# Autodesk Inventor assembly: Passion-v2
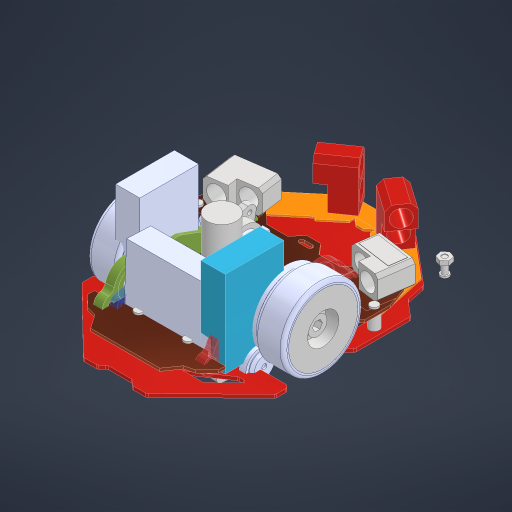
[picture p0: Inventor's stored thumbnail of the model, 512x512]
Saved by Autodesk Inventor 2023.5 (Build 275446000, 446)
## iProperties
Created: 2024-12-07
Part Number: Passion-v2
Document SubType Name: Assembly
Designer: IshiiLabHonda
Author: IshiiLabHonda
## Documents named in this file (31)
- C:\Users\IshiiLabHonda\Documents\Micromouse\Passion-v2\Inventor\Passion-v2-1\Passion-v2.iam
- C:\Users\IshiiLabHonda\Documents\Micromouse\Passion-v2\Inventor\Passion-v2-1\Readymade\Encoder-Gear_M0.3_29T.ipt
- C:\Users\IshiiLabHonda\Documents\Micromouse\Passion-v2\Inventor\Passion-v2-1\Readymade\Encoder-Gear-Spacer.ipt
- C:\Users\IshiiLabHonda\Documents\Micromouse\Passion-v2\Inventor\Passion-v2-1\Readymade\Motor-8523.ipt
- C:\Users\IshiiLabHonda\Documents\Micromouse\Passion-v2\Inventor\Passion-v2-1\Readymade\Pinion-Gear_M0.3_15T.ipt
- C:\Users\IshiiLabHonda\Documents\Micromouse\Passion-v2\Inventor\Passion-v2-1\Readymade\Spur-Gear_M0.3_71T_t2.0_D8.ipt
- C:\Users\IshiiLabHonda\Documents\Micromouse\Passion-v2\Inventor\Passion-v2-1\Readymade\Tire-MZW39-40.ipt
- C:\Users\IshiiLabHonda\Documents\Micromouse\Passion-v2\Inventor\Passion-v2-1\Readymade\Wheel_MZH131W-N2.ipt
- C:\Users\IshiiLabHonda\Documents\Micromouse\Passion-v2\Inventor\Passion-v2-1\Common\spacer_inwheel_1.1.ipt
- C:\Users\IshiiLabHonda\Documents\Micromouse\Passion-v2\Inventor\Passion-v2-1\Common\bearing_SMR63ZZ.ipt
- C:\Users\IshiiLabHonda\Documents\Micromouse\Passion-v2\Inventor\Passion-v2-1\Common\M3_bolt.ipt
- C:\Users\IshiiLabHonda\Documents\Micromouse\Passion-v2\Inventor\Passion-v2-1\Readymade\Encoder-7S-400-2MC-50-00E.ipt
- C:\Users\IshiiLabHonda\Documents\Micromouse\Passion-v2\Inventor\Passion-v2-1\Readymade\Motor-8520.ipt
- C:\Users\IshiiLabHonda\Documents\Micromouse\Passion-v2\Inventor\Passion-v2-1\Origin\encoderauxiliary.ipt
- C:\Users\IshiiLabHonda\Documents\Micromouse\Passion-v2\Inventor\Passion-v2-1\Origin\motorauxiliary.ipt
- C:\Users\IshiiLabHonda\Documents\Micromouse\Passion-v2\Inventor\Passion-v2-1\Origin\fan.ipt
- C:\Users\IshiiLabHonda\Documents\Micromouse\Passion-v2\Inventor\Passion-v2-1\Origin\motormount.ipt
- C:\Users\IshiiLabHonda\Documents\Micromouse\Passion-v2\Inventor\Passion-v2-2\Common\Li-Po_JJRC-150mAh.ipt
- C:\Users\IshiiLabHonda\Documents\Micromouse\Passion-v2\Inventor\Passion-v2-1\Origin\chassis.ipt
- C:\Users\IshiiLabHonda\Documents\Micromouse\Passion-v2\Inventor\Passion-v2-1\Origin\sensorholder_2.ipt
- C:\Users\IshiiLabHonda\Documents\Micromouse\Passion-v2\Inventor\Passion-v2-1\Origin\circuit.ipt
- C:\Users\IshiiLabHonda\Documents\Micromouse\Passion-v2\Inventor\Passion-v2-1\Common\spacer_m1.6_circuit.ipt
- C:\Users\IshiiLabHonda\Documents\Micromouse\Passion-v2\Inventor\Passion-v2-1\Common\m1.6_2_なべ小ねじ0番.ipt
- C:\Users\IshiiLabHonda\Documents\Micromouse\Passion-v2\Inventor\Passion-v2-1\Origin\sensorcircuit.ipt
- C:\Users\IshiiLabHonda\Documents\Micromouse\Passion-v2\Inventor\Passion-v2-1\Origin\sensorholder_3.ipt
- C:\Users\IshiiLabHonda\Documents\Micromouse\Passion-v2\Inventor\Passion-v2-1\Origin\fanauxiliary.ipt
- C:\Users\IshiiLabHonda\Documents\Micromouse\Passion-v2\Inventor\Passion-v2-1\Common\m1.6_3_なべ小ねじ0番.ipt
- C:\Users\IshiiLabHonda\Documents\Micromouse\Passion-v2\Inventor\Passion-v2-1\Common\m1.6_4_なべ小ねじ0番.ipt
- C:\Users\IshiiLabHonda\Documents\Micromouse\Passion-v2\Inventor\Passion-v2-1\Common\m1.6_nut.ipt
- C:\Users\IshiiLabHonda\Documents\Micromouse\Passion-v2\Inventor\Passion-v2-1\Common\m1.6_5_なべ小ねじ0番.ipt
- C:\Users\IshiiLabHonda\Documents\Micromouse\Passion-v2\Inventor\Passion-v2-1\Common\spacer-outwheel-m3-1.ipt
## Components (70 placed, 30 different names)
1. Motor-8520:1 — メイト:234, メイト:235, メイト:239
2. fan:1 — メイト:235, メイト:236, メイト:237
3. Encoder-Gear_M0.3_29T:2
4. Encoder-Gear-Spacer:2 — メイト:147
5. Motor-8523:2 — メイト:148, メイト:150, メイト:267
6. Pinion-Gear_M0.3_15T:2 — メイト:150, フラッシュ:23
7. Spur-Gear_M0.3_71T_t2.0_D8:2 — フラッシュ:23, メイト:290
8. Tire-MZW39-40:2
9. Wheel_MZH131W-N2:2
10. spacer_inwheel_1.1:2
11. bearing_SMR63ZZ:3
12. bearing_SMR63ZZ:4 — メイト:139
13. M3_bolt:2 — メイト:136, メイト:139, メイト:284
14. Encoder-7S-400-2MC-50-00E:2 — メイト:147, メイト:243, メイト:264
15. encoderauxiliary:2 — メイト:143, メイト:145, メイト:243
16. motorauxiliary:2 — メイト:140, メイト:142, メイト:148
17. motormount:2 — メイト:152, メイト:154, メイト:156, メイト:159, メイト:219, メイト:224, メイト:225, メイト:266, メイト:287, メイト:288
18. Li-Po_JJRC-150mAh:2
19. Encoder-Gear_M0.3_29T:3 — フラッシュ:25
20. Encoder-Gear-Spacer:3 — メイト:265
21. Motor-8523:3 — メイト:155, メイト:156
22. Pinion-Gear_M0.3_15T:3 — フラッシュ:24
23. Spur-Gear_M0.3_71T_t2.0_D8:3 — メイト:161, メイト:162, フラッシュ:24, フラッシュ:25, メイト:289
24. Tire-MZW39-40:3
25. Wheel_MZH131W-N2:3 — メイト:161, メイト:162
26. spacer_inwheel_1.1:3
27. bearing_SMR63ZZ:5
28. bearing_SMR63ZZ:6 — メイト:171, メイト:172
29. M3_bolt:3 — メイト:171, メイト:172, メイト:286, メイト:288
30. Encoder-7S-400-2MC-50-00E:3 — メイト:160, メイト:265, メイト:266
31. encoderauxiliary:3 — メイト:159, メイト:160, メイト:219
32. motorauxiliary:3 — メイト:152, メイト:154, メイト:155
33. motormount:3 — メイト:136, メイト:140, メイト:142, メイト:143, メイト:145, メイト:222, メイト:223, メイト:264, メイト:267, メイト:285
34. chassis:1 — メイト:177, メイト:181, メイト:182, メイト:192, メイト:195, メイト:201, メイト:206, フラッシュ:26, メイト:211, メイト:222, メイト:223, メイト:224, メイト:225, メイト:226, メイト:227, メイト:229, メイト:236, メイト:237, メイト:247, メイト:248, フラッシュ:27, メイト:255, メイト:261, メイト:263, メイト:275, メイト:278, メイト:280, メイト:281, メイト:283
35. sensorholder_2:2 — フラッシュ:27
36. sensorholder_2:4 — フラッシュ:26
37. circuit:1 — メイト:178, メイト:180, メイト:191, メイト:193, メイト:199, メイト:200, メイト:205, メイト:207, メイト:209, メイト:210, メイト:212, メイト:218, メイト:231, メイト:238, メイト:239, メイト:240, メイト:252, メイト:254, メイト:257, メイト:260, メイト:262, フラッシュ:269, フラッシュ:270, フラッシュ:273, メイト:291, フラッシュ:274
38. spacer_m1.6_circuit:1 — メイト:177, メイト:178, メイト:210
39. m1.6_2_なべ小ねじ0番:1 — メイト:180, メイト:218
40. m1.6_2_なべ小ねじ0番:2 — メイト:181, メイト:182
41. spacer_m1.6_circuit:2 — メイト:192, メイト:193, メイト:194, メイト:255
42. m1.6_2_なべ小ねじ0番:3 — メイト:191, メイト:212
43. m1.6_2_なべ小ねじ0番:4 — メイト:194, メイト:195
44. spacer_m1.6_circuit:3 — メイト:197, メイト:198, メイト:200, メイト:209, メイト:211
45. m1.6_2_なべ小ねじ0番:5 — メイト:197, メイト:199
46. m1.6_2_なべ小ねじ0番:6 — メイト:198, メイト:201
47. spacer_m1.6_circuit:4 — メイト:205
48. m1.6_2_なべ小ねじ0番:7 — メイト:207
49. m1.6_2_なべ小ねじ0番:8 — メイト:206
50. sensorcircuit:1 — メイト:247, メイト:248, メイト:271, メイト:273, メイト:274, メイト:279
51. sensorholder_3:1 — メイト:240, フラッシュ:269, フラッシュ:270
52. spacer_m1.6_circuit:5 — メイト:226, メイト:229, メイト:230
53. m1.6_2_なべ小ねじ0番:9 — メイト:230, メイト:231
54. m1.6_2_なべ小ねじ0番:10 — メイト:227, メイト:283
55. fanauxiliary:1 — メイト:234, メイト:238, メイト:252, メイト:253, メイト:256
56. m1.6_3_なべ小ねじ0番:1 — メイト:253, メイト:254
57. m1.6_3_なべ小ねじ0番:2 — メイト:256, メイト:257
58. spacer_m1.6_circuit:6 — メイト:260, メイト:261
59. m1.6_2_なべ小ねじ0番:11 — メイト:262
60. m1.6_2_なべ小ねじ0番:12 — メイト:263
61. m1.6_nut:1 — メイト:271, メイト:282
62. m1.6_4_なべ小ねじ0番:2 — メイト:273, メイト:275
63. m1.6_nut:2 — メイト:274
64. m1.6_nut:3 — メイト:278, メイト:279
65. m1.6_5_なべ小ねじ0番:1 — メイト:280, メイト:281, メイト:282
66. spacer-outwheel-m3-1:1 — メイト:284, メイト:285, メイト:290
67. spacer-outwheel-m3-1:2 — メイト:286, メイト:287, メイト:289
68. sensorholder_3:2 — フラッシュ:273, メイト:291, フラッシュ:274
69. Li-Po_JJRC-150mAh:3
70. Li-Po_JJRC-150mAh:4
## Relationships (133: Mate 118, Flush 14, Tangent 1)
- [Mate]: Encoder-Gear_M0.3_29T:2 ↔ Encoder-Gear-Spacer:2
- [Mate]: Encoder-Gear_M0.3_29T:2 ↔ Encoder-Gear-Spacer:2
- [Mate]: Spur-Gear_M0.3_71T_t2.0_D8:2 ↔ Wheel_MZH131W-N2:2
- [Mate]: Spur-Gear_M0.3_71T_t2.0_D8:2 ↔ Wheel_MZH131W-N2:2
- [Mate]: Tire-MZW39-40:2 ↔ Wheel_MZH131W-N2:2
- [Flush]: Tire-MZW39-40:2 ↔ Wheel_MZH131W-N2:2
- [Mate]: Wheel_MZH131W-N2:2 ↔ bearing_SMR63ZZ:3
- [Mate]: spacer_inwheel_1.1:2 ↔ bearing_SMR63ZZ:3
- [Mate]: bearing_SMR63ZZ:3 ↔ bearing_SMR63ZZ:4
- [Mate]: spacer_inwheel_1.1:2 ↔ bearing_SMR63ZZ:4
- [Mate]: spacer_inwheel_1.1:2 ↔ bearing_SMR63ZZ:3
- [Flush]: Wheel_MZH131W-N2:2 ↔ bearing_SMR63ZZ:3
- [Flush]: Encoder-Gear_M0.3_29T:2 ↔ Spur-Gear_M0.3_71T_t2.0_D8:2
- [Tangent] (0.1 mm): Encoder-Gear_M0.3_29T:2 ↔ Spur-Gear_M0.3_71T_t2.0_D8:2
- [Mate]: Encoder-Gear_M0.3_29T:3 ↔ Encoder-Gear-Spacer:3
- [Mate]: Encoder-Gear_M0.3_29T:3 ↔ Encoder-Gear-Spacer:3
- [Mate]: Tire-MZW39-40:3 ↔ Wheel_MZH131W-N2:3
- [Flush]: Tire-MZW39-40:3 ↔ Wheel_MZH131W-N2:3
- [Mate]: Wheel_MZH131W-N2:3 ↔ bearing_SMR63ZZ:5
- [Mate]: spacer_inwheel_1.1:3 ↔ bearing_SMR63ZZ:5
- [Mate]: bearing_SMR63ZZ:5 ↔ bearing_SMR63ZZ:6
- [Mate]: spacer_inwheel_1.1:3 ↔ bearing_SMR63ZZ:6
- [Mate]: spacer_inwheel_1.1:3 ↔ bearing_SMR63ZZ:5
- [Flush]: Wheel_MZH131W-N2:3 ↔ bearing_SMR63ZZ:5
- [Mate]: Motor-8523:3 ↔ Pinion-Gear_M0.3_15T:3
- メイト:136 [Mate]: M3_bolt:2 ↔ motormount:3
- メイト:139 [Mate]: bearing_SMR63ZZ:4 ↔ M3_bolt:2
- メイト:140 [Mate]: motorauxiliary:2 ↔ motormount:3
- メイト:142 [Mate]: motorauxiliary:2 ↔ motormount:3
- メイト:143 [Mate]: encoderauxiliary:2 ↔ motormount:3
- メイト:145 [Mate]: encoderauxiliary:2 ↔ motormount:3
- メイト:147 [Mate]: Encoder-Gear-Spacer:2 ↔ Encoder-7S-400-2MC-50-00E:2
- メイト:148 [Mate]: Motor-8523:2 ↔ motorauxiliary:2
- メイト:150 [Mate]: Motor-8523:2 ↔ Pinion-Gear_M0.3_15T:2
- フラッシュ:23 [Flush]: Pinion-Gear_M0.3_15T:2 ↔ Spur-Gear_M0.3_71T_t2.0_D8:2
- メイト:152 [Mate]: motormount:2 ↔ motorauxiliary:3
- メイト:154 [Mate]: motormount:2 ↔ motorauxiliary:3
- メイト:155 [Mate]: Motor-8523:3 ↔ motorauxiliary:3
- メイト:156 [Mate]: motormount:2 ↔ Motor-8523:3
- メイト:159 [Mate]: motormount:2 ↔ encoderauxiliary:3
- メイト:160 [Mate]: Encoder-7S-400-2MC-50-00E:3 ↔ encoderauxiliary:3
- メイト:161 [Mate]: Spur-Gear_M0.3_71T_t2.0_D8:3 ↔ Wheel_MZH131W-N2:3
- メイト:162 [Mate]: Spur-Gear_M0.3_71T_t2.0_D8:3 ↔ Wheel_MZH131W-N2:3
- フラッシュ:24 [Flush]: Pinion-Gear_M0.3_15T:3 ↔ Spur-Gear_M0.3_71T_t2.0_D8:3
- フラッシュ:25 [Flush]: Encoder-Gear_M0.3_29T:3 ↔ Spur-Gear_M0.3_71T_t2.0_D8:3
- メイト:171 [Mate]: bearing_SMR63ZZ:6 ↔ M3_bolt:3
- メイト:172 [Mate]: bearing_SMR63ZZ:6 ↔ M3_bolt:3
- メイト:177 [Mate]: chassis:1 ↔ spacer_m1.6_circuit:1
- メイト:178 [Mate]: circuit:1 ↔ spacer_m1.6_circuit:1
- メイト:180 [Mate]: circuit:1 ↔ m1.6_2_なべ小ねじ0番:1
- メイト:181 [Mate]: chassis:1 ↔ m1.6_2_なべ小ねじ0番:2
- メイト:182 [Mate]: chassis:1 ↔ m1.6_2_なべ小ねじ0番:2
- メイト:191 [Mate]: circuit:1 ↔ m1.6_2_なべ小ねじ0番:3
- メイト:192 [Mate]: chassis:1 ↔ spacer_m1.6_circuit:2
- メイト:193 [Mate]: circuit:1 ↔ spacer_m1.6_circuit:2
- メイト:194 [Mate]: spacer_m1.6_circuit:2 ↔ m1.6_2_なべ小ねじ0番:4
- メイト:195 [Mate]: chassis:1 ↔ m1.6_2_なべ小ねじ0番:4
- メイト:197 [Mate]: spacer_m1.6_circuit:3 ↔ m1.6_2_なべ小ねじ0番:5
- メイト:198 [Mate]: spacer_m1.6_circuit:3 ↔ m1.6_2_なべ小ねじ0番:6
- メイト:199 [Mate]: circuit:1 ↔ m1.6_2_なべ小ねじ0番:5
- メイト:200 [Mate]: circuit:1 ↔ spacer_m1.6_circuit:3
- メイト:201 [Mate]: chassis:1 ↔ m1.6_2_なべ小ねじ0番:6
- [Mate]: spacer_m1.6_circuit:4 ↔ m1.6_2_なべ小ねじ0番:7
- [Mate]: spacer_m1.6_circuit:4 ↔ m1.6_2_なべ小ねじ0番:8
- メイト:205 [Mate]: circuit:1 ↔ spacer_m1.6_circuit:4
- メイト:206 [Mate]: chassis:1 ↔ m1.6_2_なべ小ねじ0番:8
- メイト:207 [Mate]: circuit:1 ↔ m1.6_2_なべ小ねじ0番:7
- フラッシュ:26 [Flush]: chassis:1 ↔ sensorholder_2:4
- メイト:209 [Mate]: circuit:1 ↔ spacer_m1.6_circuit:3
- メイト:210 [Mate]: circuit:1 ↔ spacer_m1.6_circuit:1
- メイト:211 [Mate]: chassis:1 ↔ spacer_m1.6_circuit:3
- メイト:212 [Mate]: circuit:1 ↔ m1.6_2_なべ小ねじ0番:3
- メイト:218 [Mate]: circuit:1 ↔ m1.6_2_なべ小ねじ0番:1
- メイト:219 [Mate]: motormount:2 ↔ encoderauxiliary:3
- メイト:222 [Mate]: motormount:3 ↔ chassis:1
- メイト:223 [Mate]: motormount:3 ↔ chassis:1
- メイト:224 [Mate]: motormount:2 ↔ chassis:1
- メイト:225 [Mate]: motormount:2 ↔ chassis:1
- メイト:226 [Mate]: chassis:1 ↔ spacer_m1.6_circuit:5
- メイト:227 [Mate]: chassis:1 ↔ m1.6_2_なべ小ねじ0番:10
- メイト:229 [Mate]: chassis:1 ↔ spacer_m1.6_circuit:5
- メイト:230 [Mate]: spacer_m1.6_circuit:5 ↔ m1.6_2_なべ小ねじ0番:9
- メイト:231 [Mate]: circuit:1 ↔ m1.6_2_なべ小ねじ0番:9
- メイト:234 [Mate]: Motor-8520:1 ↔ fanauxiliary:1
- メイト:235 [Mate]: Motor-8520:1 ↔ fan:1
- メイト:236 [Mate]: fan:1 ↔ chassis:1
- メイト:237 [Mate] (0.5 mm): fan:1 ↔ chassis:1
- メイト:238 [Mate]: circuit:1 ↔ fanauxiliary:1
- メイト:239 [Mate]: Motor-8520:1 ↔ circuit:1
- メイト:240 [Mate]: circuit:1 ↔ sensorholder_3:1
- メイト:243 [Mate]: Encoder-7S-400-2MC-50-00E:2 ↔ encoderauxiliary:2
- メイト:247 [Mate]: chassis:1 ↔ sensorcircuit:1
- メイト:248 [Mate]: chassis:1 ↔ sensorcircuit:1
- フラッシュ:27 [Flush]: chassis:1 ↔ sensorholder_2:2
- メイト:252 [Mate]: circuit:1 ↔ fanauxiliary:1
- メイト:253 [Mate]: fanauxiliary:1 ↔ m1.6_3_なべ小ねじ0番:1
- メイト:254 [Mate]: circuit:1 ↔ m1.6_3_なべ小ねじ0番:1
- メイト:255 [Mate]: chassis:1 ↔ spacer_m1.6_circuit:2
- メイト:256 [Mate]: fanauxiliary:1 ↔ m1.6_3_なべ小ねじ0番:2
- メイト:257 [Mate]: circuit:1 ↔ m1.6_3_なべ小ねじ0番:2
- [Mate]: spacer_m1.6_circuit:6 ↔ m1.6_2_なべ小ねじ0番:11
- [Mate]: spacer_m1.6_circuit:6 ↔ m1.6_2_なべ小ねじ0番:12
- メイト:260 [Mate]: circuit:1 ↔ spacer_m1.6_circuit:6
- メイト:261 [Mate]: chassis:1 ↔ spacer_m1.6_circuit:6
- メイト:262 [Mate]: circuit:1 ↔ m1.6_2_なべ小ねじ0番:11
- メイト:263 [Mate]: chassis:1 ↔ m1.6_2_なべ小ねじ0番:12
- メイト:264 [Mate]: Encoder-7S-400-2MC-50-00E:2 ↔ motormount:3
- メイト:265 [Mate]: Encoder-Gear-Spacer:3 ↔ Encoder-7S-400-2MC-50-00E:3
- メイト:266 [Mate]: motormount:2 ↔ Encoder-7S-400-2MC-50-00E:3
- メイト:267 [Mate]: Motor-8523:2 ↔ motormount:3
- フラッシュ:269 [Flush]: circuit:1 ↔ sensorholder_3:1
- フラッシュ:270 [Flush]: circuit:1 ↔ sensorholder_3:1
- メイト:271 [Mate]: sensorcircuit:1 ↔ m1.6_nut:1
- [Mate]: m1.6_4_なべ小ねじ0番:2 ↔ m1.6_nut:2
- メイト:273 [Mate]: sensorcircuit:1 ↔ m1.6_4_なべ小ねじ0番:2
- メイト:274 [Mate]: sensorcircuit:1 ↔ m1.6_nut:2
- メイト:275 [Mate]: chassis:1 ↔ m1.6_4_なべ小ねじ0番:2
- メイト:278 [Mate]: chassis:1 ↔ m1.6_nut:3
- メイト:279 [Mate]: sensorcircuit:1 ↔ m1.6_nut:3
- メイト:280 [Mate]: chassis:1 ↔ m1.6_5_なべ小ねじ0番:1
- メイト:281 [Mate]: chassis:1 ↔ m1.6_5_なべ小ねじ0番:1
- メイト:282 [Mate]: m1.6_nut:1 ↔ m1.6_5_なべ小ねじ0番:1
- メイト:283 [Mate]: chassis:1 ↔ m1.6_2_なべ小ねじ0番:10
- メイト:284 [Mate]: M3_bolt:2 ↔ spacer-outwheel-m3-1:1
- メイト:285 [Mate]: motormount:3 ↔ spacer-outwheel-m3-1:1
- メイト:286 [Mate]: M3_bolt:3 ↔ spacer-outwheel-m3-1:2
- メイト:287 [Mate]: motormount:2 ↔ spacer-outwheel-m3-1:2
- メイト:288 [Mate]: motormount:2 ↔ M3_bolt:3
- メイト:289 [Mate]: Spur-Gear_M0.3_71T_t2.0_D8:3 ↔ spacer-outwheel-m3-1:2
- メイト:290 [Mate]: Spur-Gear_M0.3_71T_t2.0_D8:2 ↔ spacer-outwheel-m3-1:1
- フラッシュ:273 [Flush]: circuit:1 ↔ sensorholder_3:2
- メイト:291 [Mate]: circuit:1 ↔ sensorholder_3:2
- フラッシュ:274 [Flush]: circuit:1 ↔ sensorholder_3:2
## Named parameters: d72_d0 = 0 mm, d73_d1 = 0 mm, d74_d2 = 0 mm, d75_d3 = 0 mm, d76_d4 = 0 mm, d77_d5 = 0 mm, d78_d6 = 0 mm, d79_d7 = 0 mm, d80_d8 = 0 mm, d83_d11 = 0 mm, d84_d12 = 0 mm, d86_d14 = 0 mm, d88_d41 = 0 mm, d89_d42 = 0.1 mm, d140_d72_d0 = 0 mm, d141_d73_d1 = 0 mm, d144_d76_d4 = 0 mm, d145_d77_d5 = 0 mm, d146_d78_d6 = 0 mm, d147_d79_d7 = 0 mm, d148_d80_d8 = 0 mm, d151_d83_d11 = 0 mm, d152_d84_d12 = 0 mm, d154_d86_d14 = 0 mm, d161_d95_d70 = 0 mm, d297_d292 = 0 mm, d298_d293 = 0 mm, d357_d297_d292 = 0 mm, d358_d298_d293 = 0 mm, d374_d372 = 0 mm
